# Autodesk Inventor assembly: CableBraider
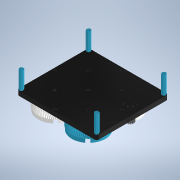
[picture p0: Inventor's stored thumbnail of the model, 180x180]
Saved by Autodesk Inventor 2021 (Build 250183000, 183)
## iProperties
Created: 2020-07-21
Part Number: CableBraider
Document SubType Name: Assembly
Designer: elmar
Author: elmar
## Documents named in this file (16)
- D:\FourWireBraidingMachine\InventorFiles\CableBraider.iam
- D:\FourWireBraidingMachine\InventorFiles\BasePlate.ipt
- D:\FourWireBraidingMachine\InventorFiles\DriveGear.ipt
- D:\FourWireBraidingMachine\InventorFiles\HornGear.ipt
- D:\FourWireBraidingMachine\InventorFiles\Standoff.ipt
- D:\FourWireBraidingMachine\InventorFiles\ReductionGearBracket.ipt
- D:\FourWireBraidingMachine\InventorFiles\ReductionGear.ipt
- D:\FourWireBraidingMachine\InventorFiles\ReductionDriveGear.ipt
- D:\FourWireBraidingMachine\InventorFiles\HornGearMirror.ipt
- D:\FourWireBraidingMachine\InventorFiles\WinderAssembly.iam
- C:\Users\elmar\OneDrive\Documents\Inventor\Content Center Files\R2021\en-US\ANSI B18.2.4.2M\ANSI B18.2.4.2M - M8x1.25 - 13.ipt
- D:\FourWireBraidingMachine\InventorFiles\Carriage.iam
- C:\Users\elmar\OneDrive\Documents\Inventor\Content Center Files\R2021\en-US\AS 1237 (2.1)\AS 1237 - 8.ipt
- C:\Users\elmar\OneDrive\Documents\Inventor\Content Center Files\R2021\en-US\AS 1112 (2)\AS 1112 - M8  Type 5.ipt
- D:\FourWireBraidingMachine\InventorFiles\GuidePlateV0.ipt
- C:\Users\elmar\OneDrive\Documents\Inventor\Content Center Files\R2021\en-US\DIN 976-1 A\DIN 976-1 - M8 x 70 - A.ipt
## Components (45 placed, 15 different names)
1. BasePlate:1 — Mate:1, Mate:2, Mate:3, Insert:3, Insert:5, Angle:1, Insert:15, Insert:17, Insert:18, Insert:19, Insert:20, Insert:21, Insert:22, Insert:23, Insert:24, Insert:25, Insert:26, Insert:28, Insert:31, Insert:38, Flush:1, Flush:2, Mate:4
2. DriveGear:1 — Insert:31, Insert:34
3. HornGear:1 — Insert:3, Angle:3, Rotation:1
4. Standoff:1 — Insert:5
5. GuidePlateV0:1 — Flush:1, Flush:2, Mate:4, Mate:5, Tangent:1, Tangent:2
6. ReductionGearBracket:1 — Angle:1, Insert:12, Insert:15, Insert:33
7. ReductionDriveGear:1 — Insert:12
8. ReductionGear:1 — Insert:33, Insert:36
9. Standoff:2 — Insert:17
10. HornGear:2 — Insert:18, Angle:3
11. HornGearMirror:1 — Insert:20, Flush:3, Angle:2
12. HornGearMirror:2 — Insert:19, Angle:2, Rotation:1
13. Standoff:3 — Insert:21
14. Standoff:4 — Insert:23
15. Standoff:5 — Insert:25
16. Standoff:6 — Insert:22
17. Standoff:7 — Insert:24
18. Standoff:8 — Insert:26
19. WinderAssembly:1 [sub-assembly]
20. ANSI B18.2.4.2M M8x1.25:2 — Insert:35
21. AS 1237 (2.1) 8:1 — Insert:34, Insert:35
22. ANSI B18.2.4.2M M8x1.25:3 — Insert:36
23. DIN 976-1 A M8 x 70:1 — Insert:39
24. ANSI B18.2.4.2M M8x1.25:1 — Insert:28, Insert:39
25. ANSI B18.2.4.2M M8x1.25:4
26. DIN 976-1 A M8 x 70:3 — Insert:40
27. DIN 976-1 A M8 x 70:4
28. DIN 976-1 A M8 x 70:5
29. DIN 976-1 A M8 x 70:6
30. AS 1112 (2) - Metric M8  Type 5:1 — Insert:38
31. AS 1112 (2) - Metric M8  Type 5:2
32. AS 1112 (2) - Metric M8  Type 5:3 — Insert:40
33. AS 1112 (2) - Metric M8  Type 5:4
34. AS 1112 (2) - Metric M8  Type 5:5
35. AS 1112 (2) - Metric M8  Type 5:6
36. AS 1112 (2) - Metric M8  Type 5:7
37. AS 1112 (2) - Metric M8  Type 5:8
38. Carriage:1 [sub-assembly] — Mate:5, Tangent:1, Tangent:2, Mate:6
39. Carriage:2 [sub-assembly]
40. Carriage:3 [sub-assembly]
41. Carriage:4 [sub-assembly]
42. Carriage:5 [sub-assembly]
43. Carriage:6 [sub-assembly]
44. Carriage:7 [sub-assembly]
45. Carriage:8 [sub-assembly]
## Component patterns: (2 elements, first: ANSI B18.2.4.2M M8x1.25:1), (4 elements, first: DIN 976-1 A M8 x 70:3), (2 elements), (4 elements, first: AS 1112 (2) - Metric M8  Type 5:1), Component Pattern 1:2 (4 elements), (2 elements), Component Pattern 5:2 (2 elements), (2 elements, first: Carriage:1), Component Pattern 4:2 (2 elements), Component Pattern 4:3 (2 elements), Component Pattern 4:4 (2 elements)
## Relationships (38: Insert 23, Mate 6, Angle 3, Flush 3, Tangent 2, RelateRotation 1)
- Mate:1: BasePlate:1
- Mate:2: BasePlate:1
- Mate:3: BasePlate:1
- Insert:3 (1 mm): BasePlate:1 ↔ HornGear:1
- Insert:5: BasePlate:1 ↔ Standoff:1
- Angle:1 (0 deg): BasePlate:1 ↔ ReductionGearBracket:1
- Insert:12 (1 mm): ReductionGearBracket:1 ↔ ReductionDriveGear:1
- Insert:15: BasePlate:1 ↔ ReductionGearBracket:1
- Insert:17: BasePlate:1 ↔ Standoff:2
- Insert:18 (1 mm): BasePlate:1 ↔ HornGear:2
- Insert:19 (1 mm): BasePlate:1 ↔ HornGearMirror:2
- Insert:20 (1 mm): BasePlate:1 ↔ HornGearMirror:1
- Insert:21: BasePlate:1 ↔ Standoff:3
- Insert:22: BasePlate:1 ↔ Standoff:6
- Insert:23: BasePlate:1 ↔ Standoff:4
- Insert:24: BasePlate:1 ↔ Standoff:7
- Insert:25: BasePlate:1 ↔ Standoff:5
- Insert:26: BasePlate:1 ↔ Standoff:8
- Insert:28: BasePlate:1 ↔ ANSI B18.2.4.2M M8x1.25:1
- Insert:31 (1 mm): BasePlate:1 ↔ DriveGear:1
- Insert:33 (1 mm): ReductionGearBracket:1 ↔ ReductionGear:1
- Insert:34: DriveGear:1 ↔ AS 1237 (2.1) 8:1
- Insert:35: ANSI B18.2.4.2M M8x1.25:2 ↔ AS 1237 (2.1) 8:1
- Insert:36: ReductionGear:1 ↔ ANSI B18.2.4.2M M8x1.25:3
- Insert:38: BasePlate:1 ↔ AS 1112 (2) - Metric M8  Type 5:1
- Insert:39: DIN 976-1 A M8 x 70:1 ↔ ANSI B18.2.4.2M M8x1.25:1
- Insert:40: DIN 976-1 A M8 x 70:3 ↔ AS 1112 (2) - Metric M8  Type 5:3
- Flush:1: BasePlate:1 ↔ GuidePlateV0:1
- Flush:2: BasePlate:1 ↔ GuidePlateV0:1
- Mate:4 (40 mm): BasePlate:1 ↔ GuidePlateV0:1
- Mate:5: GuidePlateV0:1 ↔ Carriage:1
- Tangent:1: GuidePlateV0:1 ↔ Carriage:1
- Tangent:2: GuidePlateV0:1 ↔ Carriage:1
- Flush:3 (4 mm): HornGearMirror:1
- Mate:6: Carriage:1
- Angle:2 (0 deg): HornGearMirror:1 ↔ HornGearMirror:2
- Angle:3 (0 deg): HornGear:1 ↔ HornGear:2
- Rotation:1 [RelateRotation] (1 ul): HornGear:1 ↔ HornGearMirror:2
